# Autodesk Inventor assembly: mascon-new
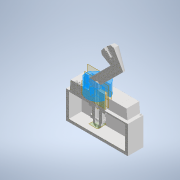
[picture p0: Inventor's stored thumbnail of the model, 180x180]
Saved by Autodesk Inventor 2022 (Build 260153000, 153)
## iProperties
Created: 2021-04-28
Part Number: mascon-new
Document SubType Name: Assembly
Designer: ben
Author: ben
## Documents named in this file (9)
- C:\Users\ben\Documents\GitHub\r68-bve-mascon\mascon-new.iam
- C:\Users\ben\Documents\GitHub\r68-bve-mascon\handle\handle.iam
- C:\Users\ben\Documents\GitHub\r68-bve-mascon\shell\shell.iam
- C:\Users\ben\Documents\GitHub\r68-bve-mascon\handle_holder.ipt
- C:\Users\ben\Documents\GitHub\r68-bve-mascon\Reverser.ipt
- C:\Users\ben\Documents\GitHub\r68-bve-mascon\handle-base\handle_base.iam
- C:\Users\ben\Documents\GitHub\r68-bve-mascon\handle_base2.ipt
- C:\Users\ben\Documents\GitHub\r68-bve-mascon\handle-base\PotAttachment.ipt
- C:\Users\ben\Documents\GitHub\r68-bve-mascon\handle-base\SpringRod.ipt
## Components (8 placed, 8 different names)
1. shell:1 [sub-assembly] — Flush:4, notch selection
2. handle_holder:1 — Mate:16
3. Reverser:1 — Flush:4
4. handle:1 [sub-assembly] — Mate:17, Flush:12, Handle Pop
5. handle_base:1 [sub-assembly] — Mate:16, Mate:17, Flush:12, Handle Pop, Mate:25, Mate:26, Mate:27, notch selection
6. handle_base2:1 — Mate:25, Mate:26, Mate:27, Mate:28
7. PotAttachment:1 — Mate:28
8. SpringRod:1
## Relationships (10: Mate 6, Flush 2, RevoluteJoint 2)
- Flush:4: shell:1 ↔ Reverser:1
- Mate:16: handle_holder:1 ↔ handle_base:1
- Mate:17: handle:1 ↔ handle_base:1
- Flush:12: handle:1 ↔ handle_base:1
- Handle Pop [RevoluteJoint]: handle:1 ↔ handle_base:1
- Mate:25: handle_base:1 ↔ handle_base2:1
- Mate:26: handle_base:1 ↔ handle_base2:1
- Mate:27: handle_base:1 ↔ handle_base2:1
- notch selection [RevoluteJoint]: shell:1 ↔ handle_base:1
- Mate:28: handle_base2:1 ↔ PotAttachment:1
